# Autodesk Inventor assembly: maze_version1
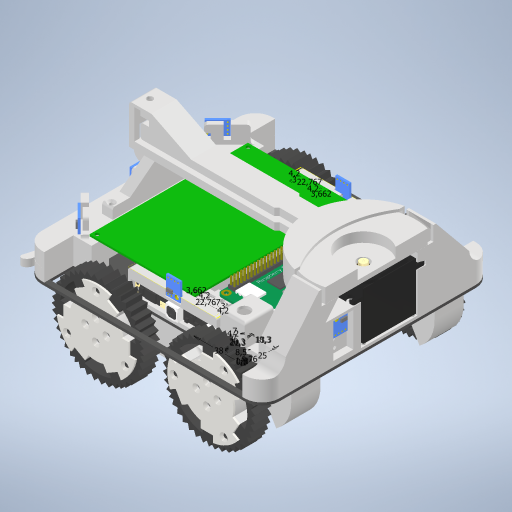
[picture p0: Inventor's stored thumbnail of the model, 512x512]
Saved by Autodesk Inventor 2023 (Build 270158000, 158)
## iProperties
Created: 2026-02-09
Part Number: maze_version1
Document SubType Name: Assembly
Designer: garin
Author: garin
## Documents named in this file (28)
- C:\Users\garin\OneDrive\Документы\maze\version1\maze_version1.iam
- C:\Users\garin\OneDrive\Документы\maze\version1\base.ipt
- C:\Users\garin\OneDrive\Документы\maze\version1\fast_battery.ipt
- C:\Users\garin\OneDrive\Документы\maze\version1\front_part_1.ipt
- C:\Users\garin\OneDrive\Документы\maze\version1\front_part_2.ipt
- C:\Users\garin\OneDrive\Документы\maze\version1\VL53L0X_TOF.ipt
- C:\Users\garin\OneDrive\Документы\maze\version1\fast_RGB.ipt
- C:\Users\garin\OneDrive\Документы\maze\version1\TCS34725 RGB sensor.ipt
- C:\Users\garin\OneDrive\Документы\maze\version1\end_cap.ipt
- C:\Users\garin\OneDrive\Документы\maze\version1\back_part.ipt
- C:\Users\garin\OneDrive\Документы\maze\version1\MG996R.ipt
- C:\Users\garin\OneDrive\Документы\maze\version1\raspberry_pi_5.ipt
- C:\Users\garin\OneDrive\Документы\maze\version1\board.ipt
- C:\Users\garin\OneDrive\Документы\maze\version1\motor_25_110RPM.ipt
- C:\Users\garin\OneDrive\Документы\maze\version1\circle.ipt
- C:\Users\garin\OneDrive\Документы\maze\version1\колёса.ipt
- C:\Users\garin\OneDrive\Документы\maze\version1\fast_motors_left.ipt
- C:\Users\garin\OneDrive\Документы\maze\version1\fast_motors_right.ipt
- C:\Users\garin\OneDrive\Документы\maze\version1\fast_akkum.ipt
- C:\Users\garin\OneDrive\Документы\maze\version1\fast_akkum2.ipt
- C:\Users\garin\OneDrive\Документы\maze\version1\system_extrad.ipt
- C:\Users\garin\OneDrive\Документы\maze\version1\fast_camera.ipt
- C:\Users\garin\OneDrive\Документы\maze\version1\Arducam USB Camera module B0431.ipt
- C:\Users\garin\OneDrive\Документы\maze\version1\TOF VL53L0X.ipt
- C:\Users\garin\OneDrive\Документы\maze\version1\wheel.iam
- C:\Users\garin\OneDrive\Документы\maze\version1\COUPLE FLANGE.ipt
- C:\Users\garin\OneDrive\Документы\maze\version1\camera.ipt
- C:\Users\garin\OneDrive\Документы\maze\version1\fast_switch.ipt
## Components (48 placed, 27 different names)
1. base:1 — Заподлицо:1, Заподлицо:2, Заподлицо:3, Заподлицо:4, С поворотом:5, Заподлицо:6, С поворотом:15, С поворотом:19, Заподлицо:10, С поворотом:21, Заподлицо:11, Заподлицо:12, Заподлицо:14, С поворотом:27, С поворотом:47, Заподлицо:15
2. fast_battery:1 — Заподлицо:1
3. front_part_1:1 — Заподлицо:2, С поворотом:6, Заподлицо:5, С поворотом:10, С поворотом:21
4. front_part_2:1 — Заподлицо:3, Заподлицо:4, С поворотом:6, С поворотом:7, С поворотом:8, С поворотом:11, С поворотом:14, С поворотом:28, С поворотом:29
5. fast_RGB:1 — С поворотом:5, С поворотом:9
6. VL53L0X_TOF:1 — С поворотом:7
7. VL53L0X_TOF:2 — С поворотом:8
8. TCS34725 RGB sensor:1 — С поворотом:9
9. end_cap:1 — Заподлицо:5
10. end_cap:2 — С поворотом:10
11. VL53L0X_TOF:3 — С поворотом:11
12. back_part:1 — Заподлицо:6, С поворотом:15, С поворотом:16, С поворотом:17, С поворотом:20, С поворотом:22, С поворотом:30
13. MG996R:1 — С поворотом:16, Заподлицо:7, Заподлицо:9
14. raspberry_pi_5:1 — С поворотом:17
15. board:1 — С поворотом:14
16. motor_25_110RPM:2 — С поворотом:36
17. motor_25_110RPM:3 — С поворотом:33
18. motor_25_110RPM:4 — С поворотом:34
19. motor_25_110RPM:5 — С поворотом:35
20. circle:1 — Заподлицо:7, Заподлицо:9, Заподлицо:13
21. колёса:1
22. fast_motors_left:1 — С поворотом:27
23. fast_motors_right:1 — С поворотом:19
24. VL53L0X_TOF:4 — С поворотом:20
25. fast_akkum:1 — Заподлицо:10
26. fast_akkum2:1 — Заподлицо:11
27. system_extrad:1 — Заподлицо:12, С поворотом:22
28. fast_camera:1 — Заподлицо:14, Жесткий:1, С поворотом:31, С поворотом:42
29. fast_camera:2 — Жесткий:2, С поворотом:47, С поворотом:48
30. Arducam USB Camera module B0431:1 — Жесткий:1
31. Arducam USB Camera module B0431:2
32. TOF VL53L0X:1
33. TOF VL53L0X:2 — С поворотом:28
34. TOF VL53L0X:3 — С поворотом:29
35. TOF VL53L0X:4 — С поворотом:30
36. TOF VL53L0X:5 — С поворотом:31
37. TOF VL53L0X:6 — С поворотом:48
38. COUPLE FLANGE:1 — С поворотом:33, С поворотом:45
39. COUPLE FLANGE:2 — С поворотом:36, С поворотом:43
40. COUPLE FLANGE:3 — С поворотом:35, С поворотом:44
41. COUPLE FLANGE:4 — С поворотом:34, С поворотом:46
42. camera:1 — Жесткий:2
43. camera:2 — С поворотом:42
44. wheel:1 [sub-assembly] — С поворотом:43
45. wheel:2 [sub-assembly] — С поворотом:46
46. wheel:3 [sub-assembly] — С поворотом:45
47. wheel:4 [sub-assembly] — С поворотом:44
48. fast_switch:1 — Заподлицо:15
## Relationships (47: RevoluteJoint 31, Flush 14, WeldJoint 2)
- Заподлицо:1 [Flush]: base:1 ↔ fast_battery:1
- Заподлицо:2 [Flush]: base:1 ↔ front_part_1:1
- Заподлицо:3 [Flush]: base:1 ↔ front_part_2:1
- Заподлицо:4 [Flush] (9 mm): base:1 ↔ front_part_2:1
- С поворотом:5 [RevoluteJoint]: base:1 ↔ fast_RGB:1
- С поворотом:6 [RevoluteJoint]: front_part_1:1 ↔ front_part_2:1
- С поворотом:7 [RevoluteJoint]: front_part_2:1 ↔ VL53L0X_TOF:1
- С поворотом:8 [RevoluteJoint]: front_part_2:1 ↔ VL53L0X_TOF:2
- С поворотом:9 [RevoluteJoint]: fast_RGB:1 ↔ TCS34725 RGB sensor:1
- Заподлицо:5 [Flush]: front_part_1:1 ↔ end_cap:1
- С поворотом:10 [RevoluteJoint]: front_part_1:1 ↔ end_cap:2
- С поворотом:11 [RevoluteJoint]: front_part_2:1 ↔ VL53L0X_TOF:3
- Заподлицо:6 [Flush]: base:1 ↔ back_part:1
- С поворотом:14 [RevoluteJoint]: front_part_2:1 ↔ board:1
- С поворотом:15 [RevoluteJoint]: base:1 ↔ back_part:1
- С поворотом:16 [RevoluteJoint]: back_part:1 ↔ MG996R:1
- С поворотом:17 [RevoluteJoint]: back_part:1 ↔ raspberry_pi_5:1
- Заподлицо:7 [Flush]: MG996R:1 ↔ circle:1
- Заподлицо:9 [Flush] (0.2 mm): MG996R:1 ↔ circle:1
- С поворотом:19 [RevoluteJoint]: base:1 ↔ fast_motors_right:1
- С поворотом:20 [RevoluteJoint]: back_part:1 ↔ VL53L0X_TOF:4
- Заподлицо:10 [Flush]: base:1 ↔ fast_akkum:1
- С поворотом:21 [RevoluteJoint]: base:1 ↔ front_part_1:1
- Заподлицо:11 [Flush]: base:1 ↔ fast_akkum2:1
- Заподлицо:12 [Flush]: base:1 ↔ system_extrad:1
- Заподлицо:13 [Flush] (-1 mm): circle:1
- С поворотом:22 [RevoluteJoint]: back_part:1 ↔ system_extrad:1
- Заподлицо:14 [Flush]: base:1 ↔ fast_camera:1
- С поворотом:27 [RevoluteJoint]: base:1 ↔ fast_motors_left:1
- Жесткий:1 [WeldJoint]: fast_camera:1 ↔ Arducam USB Camera module B0431:1
- С поворотом:28 [RevoluteJoint]: front_part_2:1 ↔ TOF VL53L0X:2
- С поворотом:29 [RevoluteJoint]: front_part_2:1 ↔ TOF VL53L0X:3
- С поворотом:30 [RevoluteJoint]: back_part:1 ↔ TOF VL53L0X:4
- С поворотом:31 [RevoluteJoint]: fast_camera:1 ↔ TOF VL53L0X:5
- С поворотом:33 [RevoluteJoint]: motor_25_110RPM:3 ↔ COUPLE FLANGE:1
- С поворотом:34 [RevoluteJoint]: motor_25_110RPM:4 ↔ COUPLE FLANGE:4
- С поворотом:35 [RevoluteJoint]: motor_25_110RPM:5 ↔ COUPLE FLANGE:3
- С поворотом:36 [RevoluteJoint]: motor_25_110RPM:2 ↔ COUPLE FLANGE:2
- С поворотом:42 [RevoluteJoint]: fast_camera:1 ↔ camera:2
- Жесткий:2 [WeldJoint]: fast_camera:2 ↔ camera:1
- С поворотом:43 [RevoluteJoint]: COUPLE FLANGE:2 ↔ wheel:1
- С поворотом:44 [RevoluteJoint]: COUPLE FLANGE:3 ↔ wheel:4
- С поворотом:45 [RevoluteJoint]: COUPLE FLANGE:1 ↔ wheel:3
- С поворотом:46 [RevoluteJoint]: COUPLE FLANGE:4 ↔ wheel:2
- С поворотом:47 [RevoluteJoint]: base:1 ↔ fast_camera:2
- С поворотом:48 [RevoluteJoint]: fast_camera:2 ↔ TOF VL53L0X:6
- Заподлицо:15 [Flush]: base:1 ↔ fast_switch:1
